# Autodesk Inventor assembly: Filament Runout Sensor Foot (1)
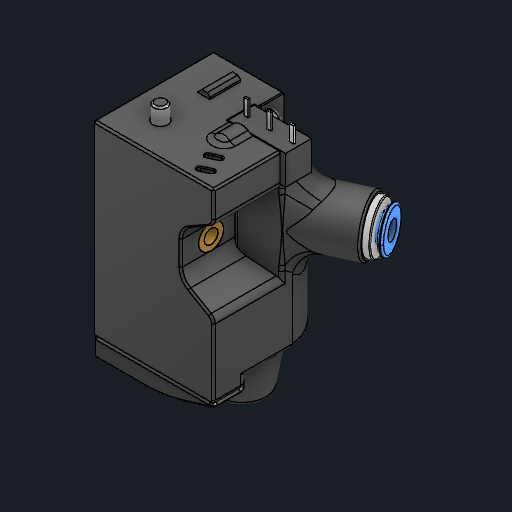
[picture p0: Inventor's stored thumbnail of the model, 512x512]
Saved by Autodesk Inventor 2026.1 (Build 301233020, 233B)
## iProperties
Created: 2025-05-09
Part Number: Filament Runout Sensor Foot (1)
Document SubType Name: Assembly
Designer: AdminForWorker
Title: Filament Runout Sensor Foot (1)
Author: AdminForWorker
## Documents named in this file (11)
- C:\Users\JoshuaEah\Documents\GitHub\Voron-0\CAD\Master Assembly\Skirt\Feet\Filament Runout Sensor Foot.iam
- C:\Users\JoshuaEah\Documents\GitHub\Voron-0\CAD\Master Assembly\Skirt\Feet\Rubber Foot.ipt
- C:\Users\JoshuaEah\Documents\GitHub\Voron-0\CAD\Master Assembly\Hardware\M2x10 Self Tapper.ipt
- C:\Users\JoshuaEah\Documents\GitHub\Voron-0\CAD\Master Assembly\Hardware\M3x40 BHCS.ipt
- C:\Users\JoshuaEah\Documents\GitHub\Voron-0\CAD\Master Assembly\Hardware\M3x10 BHCS.ipt
- C:\Users\JoshuaEah\Documents\GitHub\Voron-0\CAD\Master Assembly\Hardware\M3 Threaded Insert.ipt
- C:\Users\JoshuaEah\Documents\GitHub\Voron-0\CAD\Master Assembly\Skirt\Feet\Filament Runout Sensor Foot.ipt
- C:\Users\JoshuaEah\Documents\GitHub\Voron-0\CAD\Master Assembly\Hardware\ECAS04 Bowden Collet.ipt
- C:\Users\JoshuaEah\Documents\GitHub\Voron-0\CAD\Master Assembly\Z Axis\Parts\Omron D2F Microswitch.ipt
- C:\Users\JoshuaEah\Documents\GitHub\Voron-0\CAD\Master Assembly\Toolhead\Parts\Extruder\MR85 Bearing.ipt
- C:\Users\JoshuaEah\Documents\GitHub\Voron-0\CAD\Master Assembly\Skirt\Feet\Foot Accent.ipt
## Components (13 placed, 10 different names)
1. Filament Runout Sensor Foot:1 — Insert:4, Insert:5, Mate:1, Insert:6
2. M3 Threaded Insert:1
3. M3 Threaded Insert:2 — Insert:4
4. ECAS04 Bowden Collet:1
5. Omron D2F Microswitch:2 — Insert:5, Mate:1
6. MR85 Bearing:3
7. Rubber Foot:4
8. M2x10 Self Tapper:1
9. M2x10 Self Tapper:2
10. M2x10 Self Tapper:3
11. M3x40 BHCS:1
12. M3x10 BHCS:1
13. Foot Accent:1 — Insert:6
## Relationships (5: Insert 4, Mate 1)
- [Insert]: Omron D2F Microswitch:2 ↔ M2x10 Self Tapper:3
- Insert:4: Filament Runout Sensor Foot:1 ↔ M3 Threaded Insert:2
- Insert:5: Filament Runout Sensor Foot:1 ↔ Omron D2F Microswitch:2
- Mate:1: Filament Runout Sensor Foot:1 ↔ Omron D2F Microswitch:2
- Insert:6: Filament Runout Sensor Foot:1 ↔ Foot Accent:1
